# Autodesk Inventor assembly: ServoReductionMotor_SGER60_25
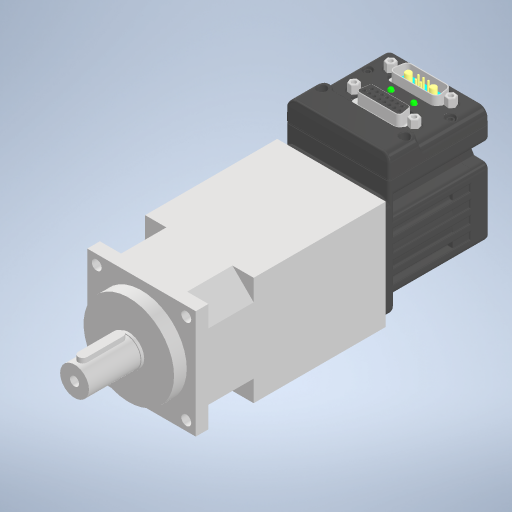
[picture p0: Inventor's stored thumbnail of the model, 512x512]
Saved by Autodesk Inventor 2023 (Build 270158000, 158)
## iProperties
Created: 2023-03-23
Part Number: ServoReductionMotor_SGER60_25
Document SubType Name: Assembly
Designer: 310611102
Mass: 1800 g
Surface Area: 357.68 cm^2
Volume: 390.373 cm^3
Density: 4.61097 g/cm^3
Author: 310611102
## Documents named in this file (2)
- C:\Users\310611102\Documents\Inventor\SSR\avionics_2023ver\actuator_system\actuator_system.iam
- C:\Users\310611102\Documents\Inventor\SSR\avionics_2023ver\actuator_system\SM23165x.ipt
## Components (1 placed, 1 different names)
1. SM23165x:1 — Flush:1, Flush:3, Mate:1
## Relationships (3: Flush 2, Mate 1)
- Flush:1: SM23165x:1
- Flush:3: SM23165x:1
- Mate:1: SM23165x:1
